# Autodesk Inventor assembly: TRAYTRAY
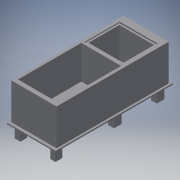
[picture p0: Inventor's stored thumbnail of the model, 180x180]
Saved by Autodesk Inventor 2019 (Build 230136000, 136)
## iProperties
Created: 2020-02-19
Part Number: TRAYTRAY
Document SubType Name: Assembly
Designer: Dell
Author: Dell
## Documents named in this file (4)
- F:\Explorers\TRAYTRAY.iam
- F:\Explorers\cstand.ipt
- F:\Explorers\collector.ipt
- F:\Explorers\tray2.ipt
## Components (3 placed, 3 different names)
1. cstand:1 — Rigid:1
2. collector:1 — Rigid:1, Rigid:2
3. tray2:1 — Rigid:2
## Relationships (2: WeldJoint 2)
- Rigid:1 [WeldJoint]: cstand:1 ↔ collector:1
- Rigid:2 [WeldJoint]: collector:1 ↔ tray2:1
